# Autodesk Inventor assembly: Assembly_Planktoscope_Lid_Screen
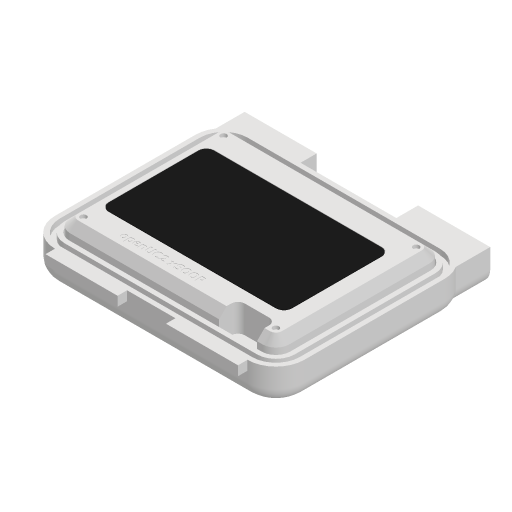
[picture p0: Inventor's stored thumbnail of the model, 512x512]
Saved by Autodesk Inventor 2024.1 (Build 281209000, 209)
## iProperties
Created: 2024-06-29
Part Number: Assembly_Planktoscope_Lid_Screen
Document SubType Name: Assembly
Designer: diederichbenedict
Mass: 1274.9 g
Surface Area: 4345.43 cm^2
Volume: 1274.9 cm^3
Density: 1 g/cm^3
Author: diederichbenedict
## Documents named in this file (4)
- C:\Users\diederichbenedict\Dropbox\Dokumente\Promotion\PROJECTS\openUC2_SOOP\INVENTOR\Workspace\Assembly_Planktoscope_Lid_Screen.iam
- C:\Users\diederichbenedict\Dropbox\Dokumente\Promotion\PROJECTS\openUC2_SOOP\INVENTOR\Workspace\00_raspberry pi display\00_raspberry pi display.ipt
- C:\Users\diederichbenedict\Dropbox\Dokumente\Promotion\PROJECTS\openUC2_SOOP\INVENTOR\Workspace\00_OutdoorCase_Type2000_toplid.ipt
- C:\Users\diederichbenedict\Dropbox\Dokumente\Promotion\PROJECTS\openUC2_SOOP\INVENTOR\Workspace\60_Planktoscope_RaspiScreenHolder_v0.ipt
## Components (3 placed, 3 different names)
1. 00_raspberry pi display:1 — Passend:1, Passend:2, Passend:3
2. 00_OutdoorCase_Type2000_toplid:1 — Passend:1, Passend:2, Passend:3, Fluchtend:1, Fluchtend:2
3. 60_Planktoscope_RaspiScreenHolder_v0:1 — Fluchtend:1, Fluchtend:2
## Relationships (5: Mate 3, Flush 2)
- Passend:1 [Mate]: 00_raspberry pi display:1 ↔ 00_OutdoorCase_Type2000_toplid:1
- Passend:2 [Mate] (5 mm): 00_raspberry pi display:1 ↔ 00_OutdoorCase_Type2000_toplid:1
- Passend:3 [Mate] (5 mm): 00_raspberry pi display:1 ↔ 00_OutdoorCase_Type2000_toplid:1
- Fluchtend:1 [Flush]: 00_OutdoorCase_Type2000_toplid:1 ↔ 60_Planktoscope_RaspiScreenHolder_v0:1
- Fluchtend:2 [Flush]: 00_OutdoorCase_Type2000_toplid:1 ↔ 60_Planktoscope_RaspiScreenHolder_v0:1
